# Autodesk Inventor assembly: Assembly1
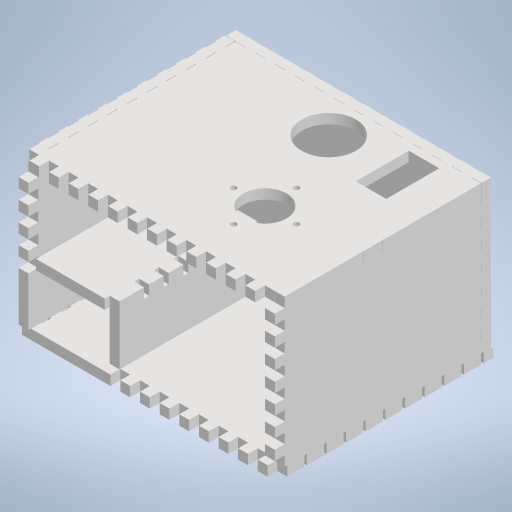
[picture p0: Inventor's stored thumbnail of the model, 512x512]
Saved by Autodesk Inventor 2024 (Build 280153000, 153)
## iProperties
Created: 2024-04-25
Part Number: Assembly1
Document SubType Name: Assembly
Designer: srika
Author: srika
## Documents named in this file (9)
- C:\Users\srika\Documents\Autodesk\Boxv3laser\Assembly1.iam
- C:\Users\srika\Documents\Autodesk\Boxv3laser\topside.ipt
- C:\Users\srika\Documents\Autodesk\Boxv3laser\frontside.ipt
- C:\Users\srika\Documents\Autodesk\Boxv3laser\backside.ipt
- C:\Users\srika\Documents\Autodesk\Boxv3laser\leftside.ipt
- C:\Users\srika\Documents\Autodesk\Boxv3laser\bottomsidesketch.ipt
- C:\Users\srika\Documents\Autodesk\Boxv3laser\middlepiecefront.ipt
- C:\Users\srika\Documents\Autodesk\Boxv3laser\middlepieceleft.ipt
- C:\Users\srika\Documents\Autodesk\Boxv3laser\middlepiecetop.ipt
## Components (8 placed, 8 different names)
1. topside:1 — Mate:1, Mate:2, Mate:6
2. frontside:1 — Mate:1
3. backside:1 — Mate:2, Mate:8
4. leftside:1 — Mate:6
5. bottomsidesketch:1 — Mate:8, Mate:9, Mate:10
6. middlepiecefront:1 — Mate:9, Mate:11
7. middlepieceleft:1 — Mate:10
8. middlepiecetop:1 — Mate:11
## Relationships (7: Mate 7)
- Mate:1: topside:1 ↔ frontside:1
- Mate:2: topside:1 ↔ backside:1
- Mate:6: topside:1 ↔ leftside:1
- Mate:8: backside:1 ↔ bottomsidesketch:1
- Mate:9: bottomsidesketch:1 ↔ middlepiecefront:1
- Mate:10: bottomsidesketch:1 ↔ middlepieceleft:1
- Mate:11: middlepiecefront:1 ↔ middlepiecetop:1
